# Autodesk Inventor assembly: mg996r_rot_into_rot
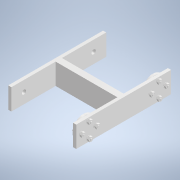
[picture p0: Inventor's stored thumbnail of the model, 180x180]
Saved by Autodesk Inventor 2021.4 (Build 254397000, 397)
## iProperties
Created: 2022-07-24
Part Number: mg996r_rot_into_rot
Document SubType Name: Assembly
Designer: isamu
Author: isamu
## Documents named in this file (6)
- D:\personal_projects\robot\inventor\2021_matlab_compat _v2\servo_rot_frame\mg996r_rot_into_rot.iam
- D:\personal_projects\robot\exports\frames\two_servo_frame_mg996r_combined.ipt
- D:\personal_projects\robot\inventor\2021_matlab_compat _v2\servo_frames\servo_handle.iam
- D:\personal_projects\robot\exports\screws\m2 washer.ipt
- D:\personal_projects\robot\exports\screws\m2 nuts.ipt
- D:\personal_projects\robot\exports\screws\m4 nuts.ipt
## Components (21 placed, 5 different names)
1. two_servo_frame_mg996r_combined:1 — Mate:1, Mate:2, Mate:3, Mate:4, Mate:5, Mate:6, Insert:1, Insert:2, Insert:3, Insert:4, Insert:5, Insert:6, Insert:7, Insert:8, Insert:17, Insert:18
2. servo_handle:1 [sub-assembly] — Mate:1, Mate:2, Mate:3
3. servo_handle:2 [sub-assembly] — Mate:4, Mate:5, Mate:6
4. m2 washer:1 — Insert:5, Insert:9
5. m2 washer:2 — Insert:2, Insert:16
6. m2 washer:3 — Insert:8, Insert:12
7. m2 washer:4 — Insert:7, Insert:11
8. m2 washer:5 — Insert:4, Insert:15
9. m2 washer:6 — Insert:6, Insert:10
10. m2 washer:7 — Insert:3, Insert:14
11. m2 washer:8 — Insert:1, Insert:13
12. m2 nuts:1 — Insert:16
13. m2 nuts:2 — Insert:13
14. m2 nuts:3 — Insert:14
15. m2 nuts:4 — Insert:15
16. m2 nuts:5 — Insert:10
17. m2 nuts:6 — Insert:11
18. m2 nuts:7 — Insert:9
19. m2 nuts:8 — Insert:12
20. m4 nuts:1 — Insert:17
21. m4 nuts:2 — Insert:18
## Relationships (24: Insert 18, Mate 6)
- Mate:1: two_servo_frame_mg996r_combined:1 ↔ servo_handle:1
- Mate:2: two_servo_frame_mg996r_combined:1 ↔ servo_handle:1
- Mate:3: two_servo_frame_mg996r_combined:1 ↔ servo_handle:1
- Mate:4: two_servo_frame_mg996r_combined:1 ↔ servo_handle:2
- Mate:5: two_servo_frame_mg996r_combined:1 ↔ servo_handle:2
- Mate:6: two_servo_frame_mg996r_combined:1 ↔ servo_handle:2
- Insert:1: two_servo_frame_mg996r_combined:1 ↔ m2 washer:8
- Insert:2: two_servo_frame_mg996r_combined:1 ↔ m2 washer:2
- Insert:3: two_servo_frame_mg996r_combined:1 ↔ m2 washer:7
- Insert:4: two_servo_frame_mg996r_combined:1 ↔ m2 washer:5
- Insert:5: two_servo_frame_mg996r_combined:1 ↔ m2 washer:1
- Insert:6: two_servo_frame_mg996r_combined:1 ↔ m2 washer:6
- Insert:7: two_servo_frame_mg996r_combined:1 ↔ m2 washer:4
- Insert:8: two_servo_frame_mg996r_combined:1 ↔ m2 washer:3
- Insert:9: m2 washer:1 ↔ m2 nuts:7
- Insert:10: m2 washer:6 ↔ m2 nuts:5
- Insert:11: m2 washer:4 ↔ m2 nuts:6
- Insert:12: m2 washer:3 ↔ m2 nuts:8
- Insert:13: m2 washer:8 ↔ m2 nuts:2
- Insert:14: m2 washer:7 ↔ m2 nuts:3
- Insert:15: m2 washer:5 ↔ m2 nuts:4
- Insert:16: m2 washer:2 ↔ m2 nuts:1
- Insert:17: two_servo_frame_mg996r_combined:1 ↔ m4 nuts:1
- Insert:18: two_servo_frame_mg996r_combined:1 ↔ m4 nuts:2
